# Autodesk Inventor assembly: ANP Filter column D1400
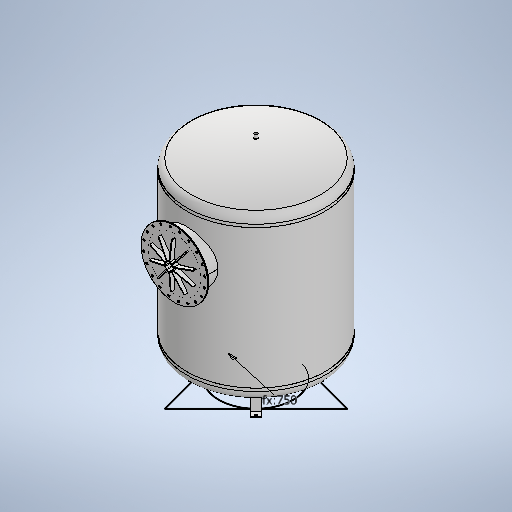
[picture p0: Inventor's stored thumbnail of the model, 512x512]
Saved by Autodesk Inventor 2025.3 (Build 293356030, 356C)
## iProperties
Created: 2025-02-13
Part Number: ANP Filter column D1400
Document SubType Name: Assembly
Designer: pokla
Mass: 522904 g
Surface Area: 229381 cm^2
Volume: 66871 cm^3
Density: 7.81959 g/cm^3
Author: pokla
Revision Number: 7
## Documents named in this file (19)
- C:\Users\admin\Yandex.Disk\home pc\Inventor\ANP--Antipayuta\ASY ANP 1400 Filter column D1400.iam
- C:\Users\admin\Yandex.Disk\home pc\Inventor\ANP--Antipayuta\ANP 1403 accses hatch flange.ipt
- C:\Users\admin\Yandex.Disk\home pc\Inventor\ANP--Antipayuta\ANP 1401 DIM Filter column D1400.ipt
- C:\Users\admin\Yandex.Disk\home pc\Inventor\ANP--Antipayuta\ANP 14031 accses hatch tube.ipt
- C:\Users\admin\Yandex.Disk\home pc\Inventor\ANP--Antipayuta\ANP 1402 SHELL D1400.ipt
- C:\Users\admin\Yandex.Disk\home pc\Inventor\ANP--Antipayuta\APN 1408 dished head.ipt
- C:\Users\admin\Yandex.Disk\home pc\Inventor\ANP--Antipayuta\Fitting G1.ipt
- C:\Users\admin\Yandex.Disk\home pc\Inventor\ANP--Antipayuta\APN 1421 charging tube.ipt
- C:\Users\admin\Yandex.Disk\home pc\Inventor\ANP--Antipayuta\ASY APN 1480 Filter legs.iam
- C:\Users\admin\Yandex.Disk\home pc\Inventor\ANP--Antipayuta\APN 1422 charging flange round.ipt
- C:\Users\admin\Yandex.Disk\home pc\Inventor\ANP--Antipayuta\sprinkler dummy.ipt
- C:\Users\admin\Yandex.Disk\home pc\Inventor\ANP--Antipayuta\ASY APN 1410 charging hatch.iam
- C:\Users\admin\Yandex.Disk\home pc\Inventor\ANP--Antipayuta\APN 1423 charging flange cup.ipt
- C:\Users\admin\Yandex.Disk\home pc\Inventor\ANP--Antipayuta\ASY APN 1430 inner elbow.iam
- C:\Users\admin\Yandex.Disk\home pc\Inventor\ANP--Antipayuta\ASY APN 1440 FDS Top elbow.iam
- C:\Users\admin\Yandex.Disk\home pc\Inventor\ANP--Antipayuta\ASY APN 1470 top funnel.iam
- C:\Users\admin\Yandex.Disk\home pc\Inventor\ANP--Antipayuta\JIS B 2312 90 Deg Long Elbow Steel 32A x Sch 40.ipt
- C:\Users\admin\Yandex.Disk\home pc\Inventor\ANP--Antipayuta\ANP 1491 accses hatch shell.ipt
- C:\Users\admin\Yandex.Disk\home pc\Inventor\ANP--Antipayuta\Fitting G1.5.ipt
## Components (60 placed, 19 different names)
1. ANP 1401 DIM Filter column D1400.ipt:1
2. APN 1421 charging tube.ipt:1 — Rigid:32
3. APN 1422 charging flange round.ipt:1 — Rigid:32, Rigid:51
4. APN 1423 charging flange cup.ipt:1 — Rigid:51
5. ASY APN 1470 top funnel.iam:1 [sub-assembly]
6. ANP 1491 accses hatch shell:1
7. APN 1408 dished head.ipt:1 — Rigid:99, Mate:5, Rigid:105, Rigid:107
8. JIS B 2312 90 Deg Long Elbow Steel 32A x Sch 40.ipt:1 — Rigid:105, Rigid:106
9. Fitting G1.5:1 — Rigid:106
10. Fitting G1:2 — Rigid:107
11. ASY APN 1430 inner elbow.iam:1 [sub-assembly] — Rigid:103
12. ASY APN 1480 Filter legs.iam:1 [sub-assembly] — Flush:2, Mate:4, Angle:1
13. ANP 14031 accses hatch tube.ipt:1 — Rigid:50, Rigid:101
14. APN 1408 dished head.ipt:2 — Rigid:100, Rigid:104
15. Fitting G1.ipt:1 — Rigid:104
16. ASY APN 1440 FDS Top elbow.iam:1 [sub-assembly] — Rigid:102
17. ANP 1402 SHELL D1400.ipt:1 — Flush:3, Flush:4, Rigid:99, Rigid:100, Rigid:101, Rigid:102, Rigid:103
18. ASY APN 1410 charging hatch.iam:1 [sub-assembly] — Rotational:4
19. ANP 1403 accses hatch flange.ipt:1 — Rotational:4, Rigid:50
20. sprinkler dummy.ipt:1
21. sprinkler dummy.ipt:2
22. sprinkler dummy.ipt:3
23. sprinkler dummy.ipt:4
24. sprinkler dummy.ipt:5
25. sprinkler dummy.ipt:6
26. sprinkler dummy.ipt:7
27. sprinkler dummy.ipt:8
28. sprinkler dummy.ipt:9
29. sprinkler dummy.ipt:10
30. sprinkler dummy.ipt:11
31. sprinkler dummy.ipt:12
32. sprinkler dummy.ipt:13
33. sprinkler dummy.ipt:14
34. sprinkler dummy.ipt:15
35. sprinkler dummy.ipt:16
36. sprinkler dummy.ipt:17
37. sprinkler dummy.ipt:18
38. sprinkler dummy.ipt:19
39. sprinkler dummy.ipt:20
40. sprinkler dummy.ipt:21
41. sprinkler dummy.ipt:22
42. sprinkler dummy.ipt:23
43. sprinkler dummy.ipt:24
44. sprinkler dummy.ipt:25
45. sprinkler dummy.ipt:26
46. sprinkler dummy.ipt:27
47. sprinkler dummy.ipt:28
48. sprinkler dummy.ipt:29
49. sprinkler dummy.ipt:30
50. sprinkler dummy.ipt:31
51. sprinkler dummy.ipt:32
52. sprinkler dummy.ipt:33
53. sprinkler dummy.ipt:34
54. sprinkler dummy.ipt:35
55. sprinkler dummy.ipt:36
56. sprinkler dummy.ipt:37
57. sprinkler dummy.ipt:38
58. sprinkler dummy.ipt:39
59. sprinkler dummy.ipt:40
60. sprinkler dummy.ipt:41
## Relationships (19: WeldJoint 12, Flush 3, Mate 2, Angle 1, RevoluteJoint 1)
- Flush:3: ANP 1402 SHELL D1400.ipt:1
- Flush:4: ANP 1402 SHELL D1400.ipt:1
- Flush:2: ASY APN 1480 Filter legs.iam:1
- Rigid:32 [WeldJoint]: APN 1421 charging tube.ipt:1 ↔ APN 1422 charging flange round.ipt:1
- Mate:4: ASY APN 1480 Filter legs.iam:1
- Angle:1 (135 deg): ASY APN 1480 Filter legs.iam:1
- Rotational:4 [RevoluteJoint]: ASY APN 1410 charging hatch.iam:1 ↔ ANP 1403 accses hatch flange.ipt:1
- Rigid:50 [WeldJoint]: ANP 14031 accses hatch tube.ipt:1 ↔ ANP 1403 accses hatch flange.ipt:1
- Rigid:51 [WeldJoint]: APN 1422 charging flange round.ipt:1 ↔ APN 1423 charging flange cup.ipt:1
- Rigid:99 [WeldJoint]: APN 1408 dished head.ipt:1 ↔ ANP 1402 SHELL D1400.ipt:1
- Rigid:100 [WeldJoint]: APN 1408 dished head.ipt:2 ↔ ANP 1402 SHELL D1400.ipt:1
- Rigid:101 [WeldJoint]: ANP 14031 accses hatch tube.ipt:1 ↔ ANP 1402 SHELL D1400.ipt:1
- Mate:5 (120 mm): APN 1408 dished head.ipt:1
- Rigid:102 [WeldJoint] (100 mm): ASY APN 1440 FDS Top elbow.iam:1 ↔ ANP 1402 SHELL D1400.ipt:1
- Rigid:103 [WeldJoint] (100 mm): ASY APN 1430 inner elbow.iam:1 ↔ ANP 1402 SHELL D1400.ipt:1
- Rigid:104 [WeldJoint]: APN 1408 dished head.ipt:2 ↔ Fitting G1.ipt:1
- Rigid:105 [WeldJoint]: APN 1408 dished head.ipt:1 ↔ JIS B 2312 90 Deg Long Elbow Steel 32A x Sch 40.ipt:1
- Rigid:106 [WeldJoint]: JIS B 2312 90 Deg Long Elbow Steel 32A x Sch 40.ipt:1 ↔ Fitting G1.5:1
- Rigid:107 [WeldJoint]: APN 1408 dished head.ipt:1 ↔ Fitting G1:2
